# Autodesk Inventor assembly: PinzettenFön2-b
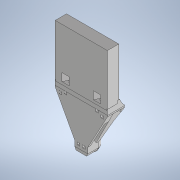
[picture p0: Inventor's stored thumbnail of the model, 180x180]
Saved by Autodesk Inventor 2020 (Build 240168000, 168)
## iProperties
Created: 2019-09-15
Part Number: PinzettenFön2-b
Document SubType Name: Assembly
Designer: rainer
Author: rainer
## Documents named in this file (5)
- N:\Projects\PinzettenFön\PinzettenFön2-b.iam
- N:\Projects\PinzettenFön\Fach2-a.ipt
- N:\Projects\PinzettenFön\Adapter_Remington.ipt
- N:\Projects\PinzettenFön\Leitung2-b.ipt
- N:\Projects\PinzettenFön\Leitung3-b.ipt
## Components (4 placed, 4 different names)
1. Leitung2-b:1 — Mate:1, Mate:2, Mate:3, Mate:8, Mate:9, Mate:10
2. Leitung3-b:1 — Mate:1, Mate:2, Mate:3, Mate:4, Mate:5, Mate:6
3. Fach2-a:1 — Mate:4, Mate:5, Mate:6
4. Adapter_Remington:1 — Mate:8, Mate:9, Mate:10
## Relationships (9: Mate 9)
- Mate:1: Leitung2-b:1 ↔ Leitung3-b:1
- Mate:2: Leitung2-b:1 ↔ Leitung3-b:1
- Mate:3: Leitung2-b:1 ↔ Leitung3-b:1
- Mate:4: Leitung3-b:1 ↔ Fach2-a:1
- Mate:5: Leitung3-b:1 ↔ Fach2-a:1
- Mate:6: Leitung3-b:1 ↔ Fach2-a:1
- Mate:8: Leitung2-b:1 ↔ Adapter_Remington:1
- Mate:9: Leitung2-b:1 ↔ Adapter_Remington:1
- Mate:10: Leitung2-b:1 ↔ Adapter_Remington:1
